# Autodesk Inventor assembly: FarmBot
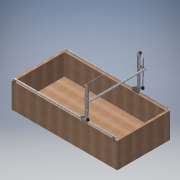
[picture p0: Inventor's stored thumbnail of the model, 180x180]
Saved by Autodesk Inventor 2017 (Build 210142000, 142)
## iProperties
Created: 2016-12-12
Part Number: FarmBot
Document SubType Name: Assembly
Designer: umr
Author: umr
## Documents named in this file (3)
- D:\SeniorProject\Models2\FarmBot.iam
- D:\SeniorProject\Models2\Elevator\Elevator.iam
- D:\SeniorProject\Models2\BedAssembly\BedAseembly.iam
## Components (2 placed, 2 different names)
1. Elevator:1 [sub-assembly] — Tangent:1, Tangent:2, Mate:1
2. BedAseembly:2 [sub-assembly] — Tangent:1, Tangent:2, Mate:1
## Relationships (3: Tangent 2, Mate 1)
- Tangent:1: Elevator:1 ↔ BedAseembly:2
- Tangent:2: Elevator:1 ↔ BedAseembly:2
- Mate:1: Elevator:1 ↔ BedAseembly:2
